# Autodesk Inventor assembly: waist
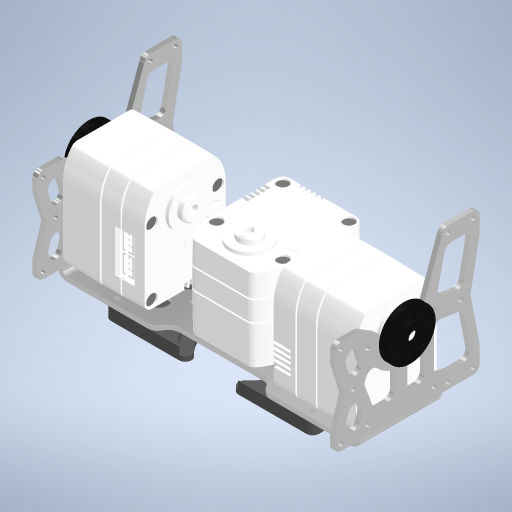
[picture p0: Inventor's stored thumbnail of the model, 512x512]
Saved by Autodesk Inventor 2024.1 (Build 281209000, 209)
## iProperties
Created: 2024-02-14
Part Number: waist
Document SubType Name: Assembly
Designer: hibik
Author: hibik
## Documents named in this file (5)
- C:\Users\hibik\Documents\Robomech\HR\Eglantyne\hard\upper_body\waist.iam
- C:\Users\hibik\Documents\Robomech\HR\Eglantyne\hard\needed_model\KRS3300モータ.ipt
- C:\Users\hibik\Documents\Robomech\HR\Eglantyne\hard\upper_body\waist_joint.ipt
- C:\Users\hibik\Documents\Robomech\HR\Eglantyne\hard\needed_model\KRS3300サーボホーン.ipt
- C:\Users\hibik\Documents\Robomech\HR\Eglantyne\hard\upper_body\waist_cover.ipt
## Components (8 placed, 4 different names)
1. waist_joint:1 — 挿入:3, 角度:3, 挿入:4, 角度:4, 挿入:7, 挿入:8, メイト:1, メイト:2, 挿入:9, 挿入:10, フラッシュ:1, フラッシュ:2
2. KRS3300モータ:2 — 挿入:3, 角度:3, 挿入:5
3. KRS3300モータ:3 — 挿入:4, 角度:4, 挿入:6
4. KRS3300サーボホーン:1 — 挿入:5
5. KRS3300サーボホーン:2 — 挿入:6
6. KRS3300モータ:4 — 挿入:7, 挿入:8
7. waist_cover:1 — メイト:1, 挿入:9, フラッシュ:2
8. waist_cover:2 — メイト:2, 挿入:10, フラッシュ:1
## Relationships (14: Insert 8, Angle 2, Mate 2, Flush 2)
- 挿入:3 [Insert]: waist_joint:1 ↔ KRS3300モータ:2
- 角度:3 [Angle] (180 deg): waist_joint:1 ↔ KRS3300モータ:2
- 挿入:4 [Insert]: waist_joint:1 ↔ KRS3300モータ:3
- 角度:4 [Angle] (180 deg): waist_joint:1 ↔ KRS3300モータ:3
- 挿入:5 [Insert] (0.3 mm): KRS3300モータ:2 ↔ KRS3300サーボホーン:1
- 挿入:6 [Insert] (0.3 mm): KRS3300モータ:3 ↔ KRS3300サーボホーン:2
- 挿入:7 [Insert]: waist_joint:1 ↔ KRS3300モータ:4
- 挿入:8 [Insert]: waist_joint:1 ↔ KRS3300モータ:4
- メイト:1 [Mate]: waist_joint:1 ↔ waist_cover:1
- メイト:2 [Mate]: waist_joint:1 ↔ waist_cover:2
- 挿入:9 [Insert]: waist_joint:1 ↔ waist_cover:1
- 挿入:10 [Insert]: waist_joint:1 ↔ waist_cover:2
- フラッシュ:1 [Flush]: waist_joint:1 ↔ waist_cover:2
- フラッシュ:2 [Flush]: waist_joint:1 ↔ waist_cover:1
